# Autodesk Inventor assembly: CessnaAssembly
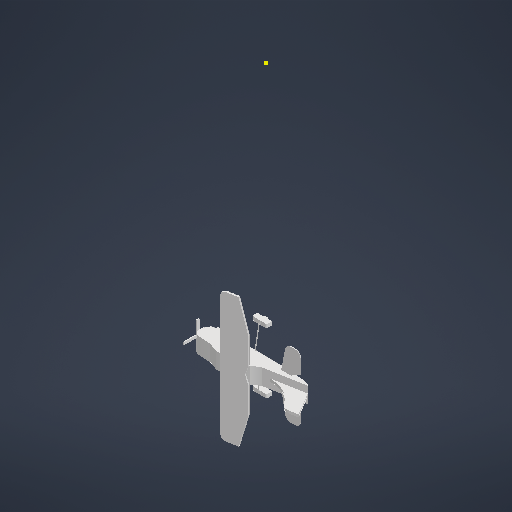
[picture p0: Inventor's stored thumbnail of the model, 512x512]
Saved by Autodesk Inventor 2027 (Build 310192060, 192F)
## iProperties
Created: 2026-07-16
Part Number: CessnaAssembly
Document SubType Name: Assembly
Designer: sunsh
Author: sunsh
## Documents named in this file (3)
- C:\Users\sunsh\OneDrive\Documents\GitHub\electric-light-utility-aircraft-multiphysics-model\models\CAD\CessnaAssembly.iam
- C:\Users\sunsh\OneDrive\Documents\GitHub\electric-light-utility-aircraft-multiphysics-model\models\CAD\CessnaAssemBody.ipt
- C:\Users\sunsh\OneDrive\Documents\GitHub\electric-light-utility-aircraft-multiphysics-model\models\CAD\CessAssemBatteryipt.ipt
## Components (2 placed, 2 different names)
1. CessnaAssemBody:1 — Mate:1
2. CessAssemBatteryipt:1 — Mate:1
## Relationships (1: Mate 1)
- Mate:1: CessnaAssemBody:1 ↔ CessAssemBatteryipt:1
